# Autodesk Inventor assembly: Walls--Basement
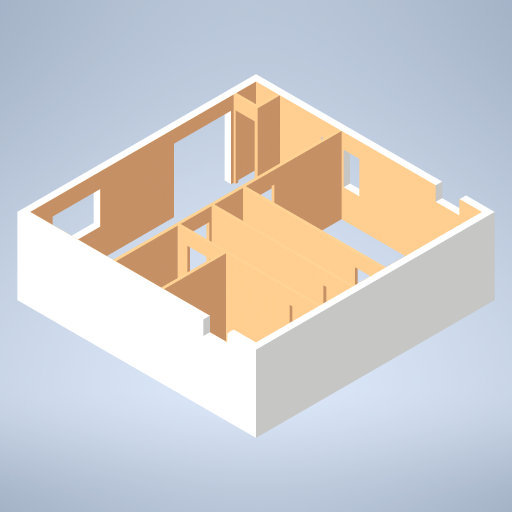
[picture p0: Inventor's stored thumbnail of the model, 512x512]
Saved by Autodesk Inventor 2024 (Build 280153000, 153)
## iProperties
Created: 2023-05-13
Part Number: Walls--Basement
Document SubType Name: Assembly
Designer: Tom
Author: Tom
## Documents named in this file (3)
- C:\Users\Tom\Documents\Tom_Levers_Public_Git_Repository\Inventor\Mobility\Basement\Finished_Basement.iam
- C:\Users\Tom\Documents\Tom_Levers_Public_Git_Repository\Inventor\Mobility\Basement\Walls--Exterior.ipt
- C:\Users\Tom\Documents\Tom_Levers_Public_Git_Repository\Inventor\Mobility\Basement\Walls--Interior.ipt
## Components (2 placed, 2 different names)
1. Walls--Exterior:1 — Mate:1, Mate:2, Flush:1, Mate:3, Flush:2, Mate:4, Mate:5, Mate:6, Flush:3
2. Walls--Interior:1 — Mate:1, Mate:2, Flush:1, Mate:3, Flush:2, Mate:4, Mate:5, Mate:6, Flush:3
## Relationships (9: Mate 6, Flush 3)
- Mate:1: Walls--Exterior:1 ↔ Walls--Interior:1
- Mate:2: Walls--Exterior:1 ↔ Walls--Interior:1
- Flush:1: Walls--Exterior:1 ↔ Walls--Interior:1
- Mate:3: Walls--Exterior:1 ↔ Walls--Interior:1
- Flush:2: Walls--Exterior:1 ↔ Walls--Interior:1
- Mate:4: Walls--Exterior:1 ↔ Walls--Interior:1
- Mate:5: Walls--Exterior:1 ↔ Walls--Interior:1
- Mate:6: Walls--Exterior:1 ↔ Walls--Interior:1
- Flush:3: Walls--Exterior:1 ↔ Walls--Interior:1
